# Autodesk Inventor assembly: MZCAT_3
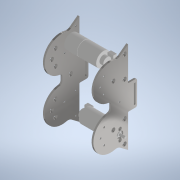
[picture p0: Inventor's stored thumbnail of the model, 180x180]
Saved by Autodesk Inventor 2022 (Build 260153000, 153)
## iProperties
Created: 2024-11-04
Part Number: MZCAT_3
Document SubType Name: Assembly
Designer: Andrey
Author: Andrey
## Documents named in this file (47)
- C:\Users\Andrey\Documents\Git\MZCAT_2024\MZCAT_3.iam
- C:\Users\Andrey\Documents\Git\MZCAT_2024\akkum_plate.ipt
- C:\Users\Andrey\Documents\Git\MZCAT_2024\base plate.ipt
- C:\Users\Andrey\Documents\Git\MZCAT_2024\base.ipt
- C:\Users\Andrey\Documents\Git\MZCAT_2024\bearing 37x25x7.ipt
- C:\Users\Andrey\Documents\Git\MZCAT_2024\CAT_protector.ipt
- C:\Users\Andrey\Documents\Git\MZCAT_2024\CAT_slave_wheel.ipt
- C:\Users\Andrey\Documents\Git\MZCAT_2024\CAT_wheel.ipt
- C:\Users\Andrey\Documents\Git\MZCAT_2024\commutationCATboard.ipt
- C:\Users\Andrey\Documents\Git\MZCAT_2024\labik.ipt
- C:\Users\Andrey\Documents\Git\MZCAT_2024\lidar_krestovina.ipt
- C:\Users\Andrey\Documents\Git\MZCAT_2024\lidar_krestovina_base.ipt
- C:\Users\Andrey\Documents\Git\MZCAT_2024\lidar_shatun_main.ipt
- C:\Users\Andrey\Documents\Git\MZCAT_2024\lidar_shatun_main2.ipt
- C:\Users\Andrey\Documents\Git\MZCAT_2024\Linit Switch.ipt
- C:\Users\Andrey\Documents\Git\MZCAT_2024\magazine.ipt
- C:\Users\Andrey\Documents\Git\MZCAT_2024\magazine_fixator.ipt
- C:\Users\Andrey\Documents\Git\MZCAT_2024\main_wheel_fixator.ipt
- C:\Users\Andrey\Documents\Git\MZCAT_2024\middle_gear_fixator.ipt
- C:\Users\Andrey\Documents\Git\MZCAT_2024\motherCATboard.ipt
- C:\Users\Andrey\Documents\Git\MZCAT_2024\motor gear.ipt
- C:\Users\Andrey\Documents\Git\MZCAT_2024\motor.ipt
- C:\Users\Andrey\Documents\Git\MZCAT_2024\OCS-D008 B.ipt
- C:\Users\Andrey\Documents\Git\MZCAT_2024\parasit_gear.ipt
- C:\Users\Andrey\Documents\Git\MZCAT_2024\plan.ipt
- C:\Users\Andrey\Documents\Git\MZCAT_2024\push-fit.ipt
- C:\Users\Andrey\Documents\Git\MZCAT_2024\vydacha_pusher.ipt
- C:\Users\Andrey\Documents\Git\MZCAT_2024\vydacha_slide.ipt
- C:\Users\Andrey\Documents\Git\MZCAT_2024\wheel_fixator.ipt
- C:\Users\Andrey\Documents\Git\MZCAT_2024\wheel_shield.ipt
- C:\Users\Andrey\Documents\Git\MZCAT_battery\FastBattery.iam
- C:\Users\Andrey\Documents\Git\MZCAT_2024\LiDAR_LD19_3D_STP_V1.0\LD19.ipt
- C:\Users\Andrey\Documents\Git\MZCAT_2024\shatun_lidar.ipt
- C:\Users\Andrey\Documents\Git\MZCAT_2024\camera fixator.ipt
- C:\Users\Andrey\Documents\Git\MZCAT_2024\camera.ipt
- C:\Users\Andrey\Documents\Git\MZCAT_2024\CM4\RaspberryPi_CM4_WithReceptacleH1.5mm.ipt
- C:\Users\Andrey\Documents\Git\MZCAT_2024\lidar lidimost.ipt
- C:\Users\Andrey\Documents\Git\MZCAT_2024\akkum_cup.ipt
- C:\Users\Andrey\Documents\Git\MZCAT_2024\concevik.ipt
- C:\Users\Andrey\Documents\Git\MZCAT_2024\concevik_mirror.ipt
- C:\Users\Andrey\Documents\Git\MZCAT_2024\karetka_lidar.ipt
- C:\Users\Andrey\Documents\Git\MZCAT_2024\2426789.ipt
- C:\Users\Andrey\Documents\Git\MZCAT_2024\camera_vision.ipt
- C:\Users\Andrey\Documents\Git\MZCAT_2024\shelka_lidar.ipt
- C:\Users\Andrey\Documents\Git\MZCAT_2024\comutation_motorboard.ipt
- C:\Users\Andrey\Documents\Git\MZCAT_2024\soldered nut.ipt
- C:\Users\Andrey\Documents\Git\MZCAT_2024\soldered nut_1,5.ipt
## Components (77 placed, 46 different names)
1. labik:1 — Совмещение:1, Заподлицо:1, Совмещение:2, Заподлицо:11, Заподлицо:12
2. plan:1 — Совмещение:1, Заподлицо:1, Совмещение:2, Совмещение:3, Совмещение:4, Совмещение:20, Заподлицо:2, Заподлицо:13, Заподлицо:47, Совмещение:49, Заподлицо:48, Заподлицо:49, Заподлицо:54, Заподлицо:56, Совмещение:78, Совмещение:84, Заподлицо:86, Совмещение:86, Заподлицо:60, Совмещение:114, Совмещение:118, Совмещение:121, Совмещение:128, Совмещение:131, Заподлицо:114, Совмещение:132, Заподлицо:145, Заподлицо:147, Совмещение:153, Совмещение:160, Совмещение:161, Совмещение:170
3. camera:3 — Заподлицо:147, Заподлицо:148, Совмещение:154, Совмещение:155, Заподлицо:149, Совмещение:160
4. camera_vision:1 — Заподлицо:148, Совмещение:154, Совмещение:155, Заподлицо:149, Совмещение:156
5. camera:4 — Совмещение:153, Заподлицо:150, Совмещение:157, Совмещение:158, Совмещение:161
6. camera_vision:2 — Заподлицо:150, Совмещение:157, Совмещение:158, Совмещение:159
7. camera:1 — Совмещение:83, Совмещение:86, Совмещение:89
8. camera:2 — Совмещение:87, Заподлицо:60, Совмещение:88
9. LD19:1
10. OCS-D008 B:2 — Совмещение:90, Совмещение:91, Совмещение:92, Заподлицо:88
11. OCS-D008 B:3 — Совмещение:93, Совмещение:94, Заподлицо:89, Совмещение:96, Заподлицо:91
12. OCS-D008 B:1 — Совмещение:113, Заподлицо:107, Совмещение:122, Совмещение:123, Заподлицо:110
13. push-fit:1 — Совмещение:100, Совмещение:104, Заподлицо:92, Совмещение:107, Совмещение:150, Заподлицо:146
14. Linit Switch:1 — Совмещение:104, Заподлицо:92, Совмещение:107, Совмещение:151
15. push-fit:2 — Совмещение:101, Совмещение:105, Совмещение:106, Совмещение:108, Совмещение:152, Заподлицо:146
16. Linit Switch:2 — Совмещение:105, Совмещение:106, Совмещение:108
17. CAT_protector:1 — Совмещение:18, Совмещение:20, Заподлицо:2, Заподлицо:90, Совмещение:95, Заподлицо:102, Заподлицо:106, Совмещение:128, Заподлицо:112, Совмещение:151, Совмещение:156, Совмещение:159, Заподлицо:151, Совмещение:184
18. akkum_cup:1 — Заподлицо:117, Совмещение:148, Совмещение:184
19. FastBattery:1 [sub-assembly] — Заподлицо:47, Совмещение:49, Совмещение:47, Совмещение:48
20. base:1 — Совмещение:3, Совмещение:4, Совмещение:5, Совмещение:6, Совмещение:7, Совмещение:8, Совмещение:9, Совмещение:10, Совмещение:13, Совмещение:14, Совмещение:15, Совмещение:16, Совмещение:18, Совмещение:79, Совмещение:80, Заподлицо:58, Заподлицо:59, Совмещение:113, Заподлицо:139, Совмещение:139, Совмещение:142, Совмещение:143, Совмещение:144, Совмещение:150, Совмещение:152, Совмещение:182, Совмещение:183
21. akkum_plate:1 — Совмещение:16, Совмещение:182, Совмещение:183
22. akkum_plate:2 — Совмещение:13, Совмещение:14, Совмещение:15, Совмещение:47
23. base plate:1 — Совмещение:5, Совмещение:9, Совмещение:10, Совмещение:30, Совмещение:31, Совмещение:32, Совмещение:33, Совмещение:34, Совмещение:35, Совмещение:40, Совмещение:51, Совмещение:54, Совмещение:185
24. base plate:2 — Совмещение:6, Совмещение:7, Совмещение:8, Совмещение:17, Совмещение:21, Совмещение:22, Совмещение:23, Совмещение:24, Совмещение:25, Совмещение:45, Совмещение:52, Совмещение:53, Совмещение:186
25. camera fixator:1 — Совмещение:79, Заподлицо:58, Совмещение:84, Совмещение:87, Совмещение:88
26. camera fixator:2 — Совмещение:80, Заподлицо:59, Совмещение:83, Заподлицо:86, Совмещение:89
27. concevik:1 — Заподлицо:139, Совмещение:139, Совмещение:142, Заподлицо:140
28. concevik_mirror:1 — Совмещение:143, Совмещение:144, Заподлицо:140
29. commutationCATboard:1 — Совмещение:48, Совмещение:100, Совмещение:101, Заподлицо:94, Совмещение:129, Совмещение:130, Заподлицо:112, Заподлицо:113, Заподлицо:117, Заподлицо:141, Совмещение:147, Совмещение:172, Совмещение:173, Совмещение:174, Совмещение:175, Совмещение:176, Совмещение:177
30. 2426789:1 — Совмещение:147, Заподлицо:145, Совмещение:148, Совмещение:149
31. motherCATboard:1 — Совмещение:118, Заподлицо:113, Совмещение:149, Совмещение:169
32. comutation_motorboard:1 — Совмещение:169, Совмещение:170, Заподлицо:151
33. RaspberryPi_CM4_WithReceptacleH1.5mm:1 — Совмещение:130, Заподлицо:141, Совмещение:178, Совмещение:179, Совмещение:180, Совмещение:181
34. soldered nut:1 — Совмещение:172
35. soldered nut:2 — Совмещение:173
36. soldered nut_1,5:1 — Совмещение:174, Совмещение:181
37. soldered nut_1,5:2 — Совмещение:175, Совмещение:180
38. soldered nut_1,5:3 — Совмещение:176, Совмещение:179
39. soldered nut_1,5:4 — Совмещение:177, Совмещение:178
40. lidar_krestovina_base:1 — Заподлицо:48, Заподлицо:49, Совмещение:64, Совмещение:65, Совмещение:93, Совмещение:94, Заподлицо:89, Совмещение:129, Совмещение:162, Совмещение:164, Совмещение:165, Совмещение:166, Совмещение:167, Совмещение:168
41. lidar_krestovina:1 — Совмещение:64, Совмещение:65, Заподлицо:54, Совмещение:90, Совмещение:91, Совмещение:98, Заподлицо:143, Заподлицо:144
42. karetka_lidar:1 — Заподлицо:143, Заподлицо:144
43. shelka_lidar:1 — Совмещение:162, Совмещение:164, Совмещение:168
44. shelka_lidar:2 — Совмещение:165, Совмещение:166, Совмещение:167
45. shatun_lidar:1 — Совмещение:92, Заподлицо:88
46. lidar_shatun_main:1 — Совмещение:96, Заподлицо:91, Совмещение:99, Совмещение:133
47. lidar_shatun_main2:1 — Совмещение:98, Совмещение:99, Совмещение:133
48. lidar lidimost:1 — Совмещение:131, Заподлицо:114, Совмещение:132
49. magazine_fixator:1 — Заподлицо:56, Совмещение:78, Заподлицо:102, Совмещение:127, Заподлицо:110, Совмещение:171
50. vydacha_pusher:1 — Совмещение:114, Совмещение:122, Совмещение:123, Совмещение:124, Совмещение:125, Совмещение:126
51. vydacha_slide:1 — Заподлицо:90, Совмещение:95, Совмещение:127
52. vydacha_pusher:2 — Совмещение:125, Совмещение:126
53. magazine:1 — Заподлицо:106, Совмещение:121, Заподлицо:107, Совмещение:124, Совмещение:171
54. motor:1 — Совмещение:40, Совмещение:41, Заподлицо:9, Совмещение:185, Заподлицо:152
55. motor:2 — Совмещение:42, Заподлицо:10, Совмещение:45, Совмещение:186, Заподлицо:152
56. motor gear:1 — Совмещение:41, Заподлицо:9
57. motor gear:2 — Совмещение:42, Заподлицо:10
58. middle_gear_fixator:1 — Совмещение:51, Совмещение:54, Совмещение:55, Заподлицо:50
59. middle_gear_fixator:2 — Совмещение:52, Совмещение:53, Совмещение:56, Заподлицо:51
60. parasit_gear:1 — Совмещение:55, Заподлицо:50
61. parasit_gear:2 — Совмещение:56, Заподлицо:51
62. main_wheel_fixator:1 — Совмещение:17, Совмещение:21, Совмещение:22, Совмещение:26, Заподлицо:4, Заподлицо:5, Совмещение:67, Совмещение:74, Совмещение:75
63. main_wheel_fixator:2 — Совмещение:30, Совмещение:31, Совмещение:32, Совмещение:37, Заподлицо:8, Заподлицо:53, Совмещение:69, Совмещение:70, Совмещение:71
64. wheel_fixator:1 — Совмещение:23, Совмещение:24, Совмещение:25, Совмещение:27, Заподлицо:3, Заподлицо:6, Совмещение:66, Совмещение:76, Совмещение:77
65. wheel_fixator:2 — Совмещение:33, Совмещение:34, Совмещение:35, Совмещение:36, Заподлицо:7, Заподлицо:52, Совмещение:68, Совмещение:72, Совмещение:73
66. bearing 37x25x7:1 — Совмещение:26, Заподлицо:4, Совмещение:28
67. bearing 37x25x7:2 — Совмещение:27, Заподлицо:3, Совмещение:29
68. bearing 37x25x7:3 — Совмещение:37, Заподлицо:8, Совмещение:58
69. bearing 37x25x7:4 — Совмещение:36, Заподлицо:7, Совмещение:57
70. CAT_wheel:1 — Совмещение:28, Заподлицо:5
71. CAT_wheel:2 — Заподлицо:53, Совмещение:58
72. CAT_slave_wheel:1 — Заподлицо:6, Совмещение:29
73. CAT_slave_wheel:2 — Совмещение:57, Заподлицо:52
74. wheel_shield:1 — Совмещение:66, Совмещение:76, Совмещение:77
75. wheel_shield:2 — Совмещение:67, Совмещение:74, Совмещение:75
76. wheel_shield:3 — Совмещение:68, Совмещение:72, Совмещение:73
77. wheel_shield:4 — Совмещение:69, Совмещение:70, Совмещение:71
## Relationships (200: Mate 147, Flush 53)
- Совмещение:1 [Mate]: labik:1 ↔ plan:1
- Заподлицо:1 [Flush]: labik:1 ↔ plan:1
- Совмещение:2 [Mate]: labik:1 ↔ plan:1
- Совмещение:3 [Mate]: plan:1 ↔ base:1
- Совмещение:4 [Mate]: plan:1 ↔ base:1
- Совмещение:5 [Mate]: base:1 ↔ base plate:1
- Совмещение:6 [Mate]: base:1 ↔ base plate:2
- Совмещение:7 [Mate]: base:1 ↔ base plate:2
- Совмещение:8 [Mate]: base:1 ↔ base plate:2
- Совмещение:9 [Mate]: base:1 ↔ base plate:1
- Совмещение:10 [Mate]: base:1 ↔ base plate:1
- Совмещение:13 [Mate]: base:1 ↔ akkum_plate:2
- Совмещение:14 [Mate]: base:1 ↔ akkum_plate:2
- Совмещение:15 [Mate] (0.1 mm): base:1 ↔ akkum_plate:2
- Совмещение:16 [Mate] (0.1 mm): base:1 ↔ akkum_plate:1
- Совмещение:17 [Mate]: base plate:2 ↔ main_wheel_fixator:1
- Совмещение:18 [Mate]: CAT_protector:1 ↔ base:1
- Совмещение:20 [Mate]: plan:1 ↔ CAT_protector:1
- Заподлицо:2 [Flush]: plan:1 ↔ CAT_protector:1
- Совмещение:21 [Mate]: base plate:2 ↔ main_wheel_fixator:1
- Совмещение:22 [Mate]: base plate:2 ↔ main_wheel_fixator:1
- Совмещение:23 [Mate]: base plate:2 ↔ wheel_fixator:1
- Совмещение:24 [Mate]: base plate:2 ↔ wheel_fixator:1
- Совмещение:25 [Mate]: base plate:2 ↔ wheel_fixator:1
- Совмещение:26 [Mate]: main_wheel_fixator:1 ↔ bearing 37x25x7:1
- Совмещение:27 [Mate]: wheel_fixator:1 ↔ bearing 37x25x7:2
- Заподлицо:3 [Flush]: wheel_fixator:1 ↔ bearing 37x25x7:2
- Заподлицо:4 [Flush]: main_wheel_fixator:1 ↔ bearing 37x25x7:1
- Совмещение:28 [Mate]: bearing 37x25x7:1 ↔ CAT_wheel:1
- Заподлицо:5 [Flush]: main_wheel_fixator:1 ↔ CAT_wheel:1
- Заподлицо:6 [Flush]: wheel_fixator:1 ↔ CAT_slave_wheel:1
- Совмещение:29 [Mate]: bearing 37x25x7:2 ↔ CAT_slave_wheel:1
- Совмещение:30 [Mate]: base plate:1 ↔ main_wheel_fixator:2
- Совмещение:31 [Mate]: base plate:1 ↔ main_wheel_fixator:2
- Совмещение:32 [Mate]: base plate:1 ↔ main_wheel_fixator:2
- Совмещение:33 [Mate]: base plate:1 ↔ wheel_fixator:2
- Совмещение:34 [Mate]: base plate:1 ↔ wheel_fixator:2
- Совмещение:35 [Mate]: base plate:1 ↔ wheel_fixator:2
- Совмещение:36 [Mate]: wheel_fixator:2 ↔ bearing 37x25x7:4
- Совмещение:37 [Mate]: main_wheel_fixator:2 ↔ bearing 37x25x7:3
- Заподлицо:7 [Flush]: wheel_fixator:2 ↔ bearing 37x25x7:4
- Заподлицо:8 [Flush]: main_wheel_fixator:2 ↔ bearing 37x25x7:3
- Совмещение:40 [Mate]: base plate:1 ↔ motor:1
- Совмещение:41 [Mate]: motor:1 ↔ motor gear:1
- Заподлицо:9 [Flush]: motor:1 ↔ motor gear:1
- Совмещение:42 [Mate]: motor:2 ↔ motor gear:2
- Заподлицо:10 [Flush]: motor:2 ↔ motor gear:2
- Совмещение:45 [Mate]: base plate:2 ↔ motor:2
- Заподлицо:11 [Flush]: labik:1
- Заподлицо:12 [Flush]: labik:1
- Заподлицо:13 [Flush]: plan:1
- Заподлицо:47 [Flush]: plan:1 ↔ FastBattery:1
- Совмещение:49 [Mate]: plan:1 ↔ FastBattery:1
- Совмещение:47 [Mate] (0.1 mm): FastBattery:1 ↔ akkum_plate:2
- Совмещение:48 [Mate] (3 mm): FastBattery:1 ↔ commutationCATboard:1
- Заподлицо:48 [Flush]: plan:1 ↔ lidar_krestovina_base:1
- Заподлицо:49 [Flush]: plan:1 ↔ lidar_krestovina_base:1
- Совмещение:51 [Mate]: base plate:1 ↔ middle_gear_fixator:1
- Совмещение:52 [Mate]: base plate:2 ↔ middle_gear_fixator:2
- Совмещение:53 [Mate]: base plate:2 ↔ middle_gear_fixator:2
- Совмещение:54 [Mate]: base plate:1 ↔ middle_gear_fixator:1
- Совмещение:55 [Mate]: middle_gear_fixator:1 ↔ parasit_gear:1
- Заподлицо:50 [Flush]: middle_gear_fixator:1 ↔ parasit_gear:1
- Совмещение:56 [Mate]: middle_gear_fixator:2 ↔ parasit_gear:2
- Заподлицо:51 [Flush]: middle_gear_fixator:2 ↔ parasit_gear:2
- Совмещение:57 [Mate]: bearing 37x25x7:4 ↔ CAT_slave_wheel:2
- Заподлицо:52 [Flush]: wheel_fixator:2 ↔ CAT_slave_wheel:2
- Заподлицо:53 [Flush]: main_wheel_fixator:2 ↔ CAT_wheel:2
- Совмещение:58 [Mate]: bearing 37x25x7:3 ↔ CAT_wheel:2
- Совмещение:64 [Mate]: lidar_krestovina_base:1 ↔ lidar_krestovina:1
- Совмещение:65 [Mate]: lidar_krestovina_base:1 ↔ lidar_krestovina:1
- Заподлицо:54 [Flush]: plan:1 ↔ lidar_krestovina:1
- Совмещение:66 [Mate]: wheel_fixator:1 ↔ wheel_shield:1
- Совмещение:67 [Mate]: main_wheel_fixator:1 ↔ wheel_shield:2
- Совмещение:68 [Mate]: wheel_fixator:2 ↔ wheel_shield:3
- Совмещение:69 [Mate]: main_wheel_fixator:2 ↔ wheel_shield:4
- Совмещение:70 [Mate]: main_wheel_fixator:2 ↔ wheel_shield:4
- Совмещение:71 [Mate]: main_wheel_fixator:2 ↔ wheel_shield:4
- Совмещение:72 [Mate]: wheel_fixator:2 ↔ wheel_shield:3
- Совмещение:73 [Mate]: wheel_fixator:2 ↔ wheel_shield:3
- Совмещение:74 [Mate]: main_wheel_fixator:1 ↔ wheel_shield:2
- Совмещение:75 [Mate]: main_wheel_fixator:1 ↔ wheel_shield:2
- Совмещение:76 [Mate]: wheel_fixator:1 ↔ wheel_shield:1
- Совмещение:77 [Mate]: wheel_fixator:1 ↔ wheel_shield:1
- Заподлицо:56 [Flush]: plan:1 ↔ magazine_fixator:1
- Совмещение:78 [Mate]: plan:1 ↔ magazine_fixator:1
- Совмещение:79 [Mate]: base:1 ↔ camera fixator:1
- Совмещение:80 [Mate]: base:1 ↔ camera fixator:2
- Заподлицо:58 [Flush]: base:1 ↔ camera fixator:1
- Заподлицо:59 [Flush]: base:1 ↔ camera fixator:2
- Совмещение:83 [Mate]: camera:1 ↔ camera fixator:2
- Совмещение:84 [Mate]: plan:1 ↔ camera fixator:1
- Заподлицо:86 [Flush]: plan:1 ↔ camera fixator:2
- Совмещение:86 [Mate]: plan:1 ↔ camera:1
- Совмещение:87 [Mate]: camera:2 ↔ camera fixator:1
- Заподлицо:60 [Flush]: plan:1 ↔ camera:2
- Совмещение:88 [Mate] (0.5 mm): camera:2 ↔ camera fixator:1
- Совмещение:89 [Mate] (0.5 mm): camera:1 ↔ camera fixator:2
- Совмещение:90 [Mate]: OCS-D008 B:2 ↔ lidar_krestovina:1
- Совмещение:91 [Mate]: OCS-D008 B:2 ↔ lidar_krestovina:1
- Совмещение:92 [Mate]: OCS-D008 B:2 ↔ shatun_lidar:1
- Заподлицо:88 [Flush]: OCS-D008 B:2 ↔ shatun_lidar:1
- Совмещение:93 [Mate]: OCS-D008 B:3 ↔ lidar_krestovina_base:1
- Совмещение:94 [Mate]: OCS-D008 B:3 ↔ lidar_krestovina_base:1
- Заподлицо:89 [Flush] (1.8 mm): OCS-D008 B:3 ↔ lidar_krestovina_base:1
- Заподлицо:90 [Flush]: CAT_protector:1 ↔ vydacha_slide:1
- Совмещение:95 [Mate] (0.048 mm): CAT_protector:1 ↔ vydacha_slide:1
- Совмещение:96 [Mate]: OCS-D008 B:3 ↔ lidar_shatun_main:1
- Заподлицо:91 [Flush]: OCS-D008 B:3 ↔ lidar_shatun_main:1
- Совмещение:98 [Mate]: lidar_krestovina:1 ↔ lidar_shatun_main2:1
- Совмещение:99 [Mate] (0.2 mm): lidar_shatun_main:1 ↔ lidar_shatun_main2:1
- Совмещение:100 [Mate]: push-fit:1 ↔ commutationCATboard:1
- Совмещение:101 [Mate]: push-fit:2 ↔ commutationCATboard:1
- Совмещение:104 [Mate]: push-fit:1 ↔ Linit Switch:1
- Совмещение:105 [Mate]: push-fit:2 ↔ Linit Switch:2
- Заподлицо:92 [Flush]: push-fit:1 ↔ Linit Switch:1
- Заподлицо:94 [Flush]: commutationCATboard:1
- Совмещение:106 [Mate]: push-fit:2 ↔ Linit Switch:2
- Совмещение:107 [Mate] (0.1 mm): push-fit:1 ↔ Linit Switch:1
- Совмещение:108 [Mate] (0.1 mm): push-fit:2 ↔ Linit Switch:2
- Совмещение:113 [Mate]: OCS-D008 B:1 ↔ base:1
- Совмещение:114 [Mate]: plan:1 ↔ vydacha_pusher:1
- Совмещение:118 [Mate]: plan:1 ↔ motherCATboard:1
- Заподлицо:102 [Flush] (0.048 mm): CAT_protector:1 ↔ magazine_fixator:1
- Заподлицо:106 [Flush]: CAT_protector:1 ↔ magazine:1
- Совмещение:121 [Mate]: plan:1 ↔ magazine:1
- Заподлицо:107 [Flush]: OCS-D008 B:1 ↔ magazine:1
- Совмещение:122 [Mate]: OCS-D008 B:1 ↔ vydacha_pusher:1
- Совмещение:123 [Mate] (0.1 mm): OCS-D008 B:1 ↔ vydacha_pusher:1
- Совмещение:124 [Mate]: vydacha_pusher:1 ↔ magazine:1
- Совмещение:125 [Mate]: vydacha_pusher:1 ↔ vydacha_pusher:2
- Совмещение:126 [Mate]: vydacha_pusher:1 ↔ vydacha_pusher:2
- Совмещение:127 [Mate] (0.3 mm): magazine_fixator:1 ↔ vydacha_slide:1
- Заподлицо:110 [Flush]: OCS-D008 B:1 ↔ magazine_fixator:1
- Совмещение:128 [Mate]: plan:1 ↔ CAT_protector:1
- Совмещение:129 [Mate] (2 mm): commutationCATboard:1 ↔ lidar_krestovina_base:1
- Совмещение:130 [Mate]: commutationCATboard:1 ↔ RaspberryPi_CM4_WithReceptacleH1.5mm:1
- Заподлицо:112 [Flush]: CAT_protector:1 ↔ commutationCATboard:1
- Заподлицо:113 [Flush]: commutationCATboard:1 ↔ motherCATboard:1
- Совмещение:131 [Mate]: plan:1 ↔ lidar lidimost:1
- Заподлицо:114 [Flush]: plan:1 ↔ lidar lidimost:1
- Совмещение:132 [Mate]: plan:1 ↔ lidar lidimost:1
- Совмещение:133 [Mate]: lidar_shatun_main:1 ↔ lidar_shatun_main2:1
- Заподлицо:117 [Flush]: akkum_cup:1 ↔ commutationCATboard:1
- Заподлицо:139 [Flush]: base:1 ↔ concevik:1
- Совмещение:139 [Mate]: base:1 ↔ concevik:1
- Совмещение:142 [Mate]: base:1 ↔ concevik:1
- Совмещение:143 [Mate]: base:1 ↔ concevik_mirror:1
- Совмещение:144 [Mate] (0.3 mm): base:1 ↔ concevik_mirror:1
- Заподлицо:140 [Flush]: concevik:1 ↔ concevik_mirror:1
- Заподлицо:141 [Flush] (1 mm): commutationCATboard:1 ↔ RaspberryPi_CM4_WithReceptacleH1.5mm:1
- Заподлицо:143 [Flush]: lidar_krestovina:1 ↔ karetka_lidar:1
- Заподлицо:144 [Flush]: lidar_krestovina:1 ↔ karetka_lidar:1
- Совмещение:147 [Mate]: commutationCATboard:1 ↔ 2426789:1
- Заподлицо:145 [Flush]: plan:1 ↔ 2426789:1
- Совмещение:148 [Mate] (1 mm): akkum_cup:1 ↔ 2426789:1
- Совмещение:149 [Mate] (0.08 mm): 2426789:1 ↔ motherCATboard:1
- Совмещение:150 [Mate]: push-fit:1 ↔ base:1
- Совмещение:151 [Mate] (0.5 mm): Linit Switch:1 ↔ CAT_protector:1
- Совмещение:152 [Mate]: push-fit:2 ↔ base:1
- Заподлицо:146 [Flush]: push-fit:1 ↔ push-fit:2
- Заподлицо:147 [Flush]: plan:1 ↔ camera:3
- Совмещение:153 [Mate]: plan:1 ↔ camera:4
- Заподлицо:148 [Flush]: camera:3 ↔ camera_vision:1
- Совмещение:154 [Mate]: camera:3 ↔ camera_vision:1
- Совмещение:155 [Mate]: camera:3 ↔ camera_vision:1
- Заподлицо:149 [Flush]: camera:3 ↔ camera_vision:1
- Совмещение:156 [Mate]: camera_vision:1 ↔ CAT_protector:1
- Заподлицо:150 [Flush]: camera:4 ↔ camera_vision:2
- Совмещение:157 [Mate]: camera:4 ↔ camera_vision:2
- Совмещение:158 [Mate]: camera:4 ↔ camera_vision:2
- Совмещение:159 [Mate]: camera_vision:2 ↔ CAT_protector:1
- Совмещение:160 [Mate]: plan:1 ↔ camera:3
- Совмещение:161 [Mate]: plan:1 ↔ camera:4
- Совмещение:162 [Mate]: lidar_krestovina_base:1 ↔ shelka_lidar:1
- Совмещение:164 [Mate] (0.5 mm): lidar_krestovina_base:1 ↔ shelka_lidar:1
- Совмещение:165 [Mate]: lidar_krestovina_base:1 ↔ shelka_lidar:2
- Совмещение:166 [Mate] (0.5 mm): lidar_krestovina_base:1 ↔ shelka_lidar:2
- Совмещение:167 [Mate] (0.2 mm): lidar_krestovina_base:1 ↔ shelka_lidar:2
- Совмещение:168 [Mate] (0.2 mm): lidar_krestovina_base:1 ↔ shelka_lidar:1
- Совмещение:169 [Mate] (4 mm): motherCATboard:1 ↔ comutation_motorboard:1
- Совмещение:170 [Mate]: plan:1 ↔ comutation_motorboard:1
- Заподлицо:151 [Flush] (10 mm): CAT_protector:1 ↔ comutation_motorboard:1
- Совмещение:171 [Mate]: magazine_fixator:1 ↔ magazine:1
- Совмещение:172 [Mate]: commutationCATboard:1 ↔ soldered nut:1
- Совмещение:173 [Mate]: commutationCATboard:1 ↔ soldered nut:2
- Совмещение:174 [Mate]: commutationCATboard:1 ↔ soldered nut_1,5:1
- Совмещение:175 [Mate]: commutationCATboard:1 ↔ soldered nut_1,5:2
- Совмещение:176 [Mate]: commutationCATboard:1 ↔ soldered nut_1,5:3
- Совмещение:177 [Mate]: commutationCATboard:1 ↔ soldered nut_1,5:4
- Совмещение:178 [Mate]: RaspberryPi_CM4_WithReceptacleH1.5mm:1 ↔ soldered nut_1,5:4
- Совмещение:179 [Mate]: RaspberryPi_CM4_WithReceptacleH1.5mm:1 ↔ soldered nut_1,5:3
- Совмещение:180 [Mate]: RaspberryPi_CM4_WithReceptacleH1.5mm:1 ↔ soldered nut_1,5:2
- Совмещение:181 [Mate]: RaspberryPi_CM4_WithReceptacleH1.5mm:1 ↔ soldered nut_1,5:1
- Совмещение:182 [Mate]: base:1 ↔ akkum_plate:1
- Совмещение:183 [Mate]: base:1 ↔ akkum_plate:1
- Совмещение:184 [Mate]: CAT_protector:1 ↔ akkum_cup:1
- Совмещение:185 [Mate]: base plate:1 ↔ motor:1
- Совмещение:186 [Mate]: base plate:2 ↔ motor:2
- Заподлицо:152 [Flush]: motor:1 ↔ motor:2
